# Autodesk Inventor assembly: omni wheel short low channel
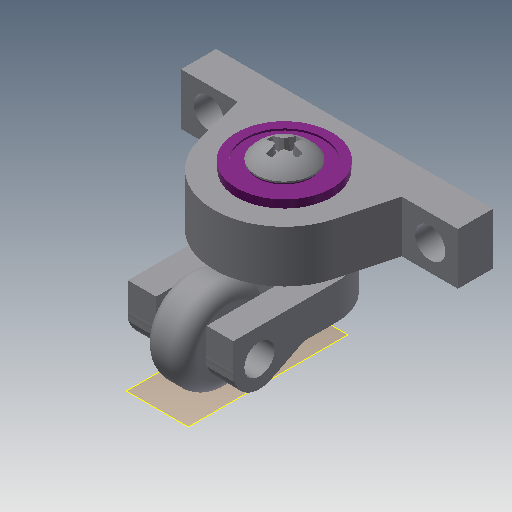
[picture p0: Inventor's stored thumbnail of the model, 512x512]
Saved by Autodesk Inventor 2018 (Build 220112000, 112)
## iProperties
Created: 2019-02-06
Part Number: omni wheel short low channel
Document SubType Name: Assembly
Designer: ball
Author: ball
## Documents named in this file (9)
- C:\FTC\FTC8863CAD\2018Robot\omni wheel short low channel.iam
- C:\FTC\FTC8863CAD\StepLibraries\Screws\6-32x.375_18-8 SS TRUSS HEAD PHILLIPS MACHINE SCREW.ipt
- C:\FTC\FTC8863CAD\2018Robot\Collector Wheel.ipt
- C:\FTC\FTC8863CAD\Actobotics\535 parts\535198.ipt
- C:\FTC\FTC8863CAD\Actobotics\633 parts\633120.ipt
- C:\FTC\FTC8863CAD\StepLibraries\Screws\6-32x.250_18-8 SS TRUSS HEAD PHILLIPS MACHINE SCREW.ipt
- C:\FTC\FTC8863CAD\Actobotics\633 parts\633104.ipt
- C:\FTC\FTC8863CAD\2018Robot\omni wheel shaft holder low channel side attach.ipt
- C:\FTC\FTC8863CAD\2018Robot\omni wheel short low channel mount.ipt
## Components (9 placed, 8 different names)
1. 6-32x.375_18-8 SS TRUSS HEAD PHILLIPS MACHINE SCREW:1 — Mate:2, Angle:1, Mate:10, Tangent:2
2. Collector Wheel:1 — Tangent:1, Tangent:2
3. 535198:1 — Mate:2, Mate:3, Mate:4, Mate:8, Mate:9
4. 535198:2 — Mate:3, Mate:4, Flush:1, Mate:5, Mate:6, Mate:12
5. 633120:1 — Flush:1, Mate:5, Mate:7
6. 6-32x.250_18-8 SS TRUSS HEAD PHILLIPS MACHINE SCREW:1 — Mate:6, Mate:7
7. 633104:1 — Mate:8, Mate:9, Mate:10, Mate:13
8. omni wheel shaft holder low channel side attach:1 — Mate:11, Mate:12, Mate:13
9. omni wheel short low channel mount:1
## Relationships (16: Mate 12, Tangent 2, Angle 1, Flush 1)
- Mate:2: 6-32x.375_18-8 SS TRUSS HEAD PHILLIPS MACHINE SCREW:1 ↔ 535198:1
- Angle:1 (0 deg): 6-32x.375_18-8 SS TRUSS HEAD PHILLIPS MACHINE SCREW:1
- Tangent:1: Collector Wheel:1
- Mate:3 (0.254 mm): 535198:1 ↔ 535198:2
- Mate:4: 535198:1 ↔ 535198:2
- Flush:1: 535198:2 ↔ 633120:1
- Mate:5: 535198:2 ↔ 633120:1
- Mate:6: 535198:2 ↔ 6-32x.250_18-8 SS TRUSS HEAD PHILLIPS MACHINE SCREW:1
- Mate:7: 633120:1 ↔ 6-32x.250_18-8 SS TRUSS HEAD PHILLIPS MACHINE SCREW:1
- Mate:8: 535198:1 ↔ 633104:1
- Mate:9: 535198:1 ↔ 633104:1
- Mate:10 (5.08 mm): 6-32x.375_18-8 SS TRUSS HEAD PHILLIPS MACHINE SCREW:1 ↔ 633104:1
- Mate:11 (13.335 mm): omni wheel shaft holder low channel side attach:1
- Tangent:2 (0.635 mm): 6-32x.375_18-8 SS TRUSS HEAD PHILLIPS MACHINE SCREW:1 ↔ Collector Wheel:1
- Mate:12: 535198:2 ↔ omni wheel shaft holder low channel side attach:1
- Mate:13: 633104:1 ↔ omni wheel shaft holder low channel side attach:1
